# Autodesk Inventor assembly: BOOM ASSEMBLY
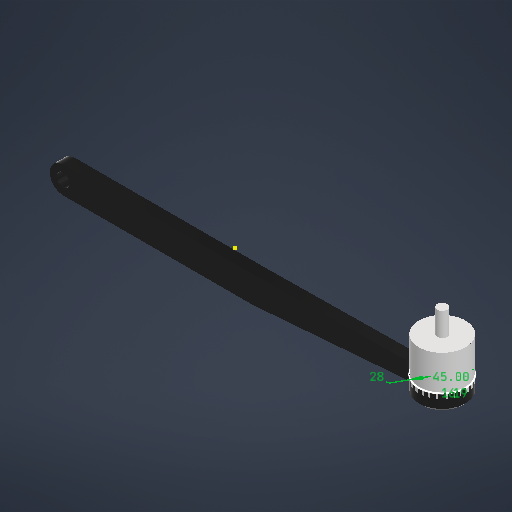
[picture p0: Inventor's stored thumbnail of the model, 512x512]
Saved by Autodesk Inventor 2025 (Build 290162010, 162A)
## iProperties
Created: 2025-05-21
Part Number: BOOM ASSEMBLY
Document SubType Name: Assembly
Designer: Jebediah Kerman
Author: Jebediah Kerman
## Documents named in this file (3)
- F:\Desktop\Projects\RTLS_VIC\CAD\BOOM ASSEMBLY.iam
- F:\Desktop\Projects\RTLS_VIC\CAD\BOOM ARM.ipt
- F:\Desktop\Projects\RTLS_VIC\CAD\MOTOR.ipt
## Components (2 placed, 2 different names)
1. BOOM ARM:1 — Mate:1, Mate:2, Mate:3
2. MOTOR:1 — Mate:1, Mate:2, Mate:3
## Relationships (3: Mate 3)
- Mate:1: BOOM ARM:1 ↔ MOTOR:1
- Mate:2: BOOM ARM:1 ↔ MOTOR:1
- Mate:3: BOOM ARM:1 ↔ MOTOR:1
